# Autodesk Inventor assembly: Ensamblaje_Final
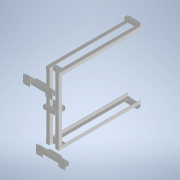
[picture p0: Inventor's stored thumbnail of the model, 180x180]
Saved by Autodesk Inventor 2020 (Build 240168000, 168)
## iProperties
Created: 2022-03-28
Part Number: Ensamblaje_Final
Document SubType Name: Assembly
Designer: aarco
Author: aarco
## Documents named in this file (8)
- C:\Users\aarco\Desktop\IDOM\REV_3\Ensamblaje_Final.iam
- C:\Users\aarco\Desktop\IDOM\REV_3\C_358_40_2.ipt
- C:\Users\aarco\Desktop\IDOM\REV_3\C_150_40_2.ipt
- C:\Users\aarco\Desktop\IDOM\REV_3\C_805_40_2.ipt
- C:\Users\aarco\Desktop\IDOM\REV_3\C_154_40_2.ipt
- C:\Users\aarco\Desktop\IDOM\REV_3\Placa_Rueda_105x85_80x60_3.ipt
- C:\Users\aarco\Desktop\IDOM\REV_3\A_992_40_4.ipt
- C:\Users\aarco\Desktop\IDOM\REV_3\C_150_40_20_2.ipt
## Components (20 placed, 7 different names)
1. C_358_40_2:1 — Rígido:16, Rígido:19, Rígido:27
2. C_358_40_2:2 — Rígido:17, Rígido:18, Rígido:26
3. C_150_40_2:1 — Rígido:1, Rígido:2
4. C_150_40_2:4 — Rígido:5
5. C_150_40_2:5 — Rígido:6
6. C_150_40_2:6 — Rígido:7
7. C_805_40_2:1 — Rígido:2, Rígido:6, Rígido:7, Rígido:22, Rígido:23
8. C_805_40_2:2 — Rígido:1, Rígido:5, Rígido:20, Rígido:21
9. C_154_40_2:1 — Rígido:24
10. C_154_40_2:2 — Rígido:25
11. Placa_Rueda_105x85_80x60_3:1 — Rígido:16
12. Placa_Rueda_105x85_80x60_3:2 — Rígido:17
13. Placa_Rueda_105x85_80x60_3:3 — Rígido:18
14. Placa_Rueda_105x85_80x60_3:4 — Rígido:19
15. A_992_40_4:1 — Rígido:20
16. A_992_40_4:2 — Rígido:22, Rígido:24
17. A_992_40_4:3 — Rígido:23, Rígido:25
18. A_992_40_4:4 — Rígido:21
19. C_150_40_20_2:1 — Rígido:26
20. C_150_40_20_2:2 — Rígido:27
## Relationships (17: WeldJoint 17)
- Rígido:1 [WeldJoint]: C_150_40_2:1 ↔ C_805_40_2:2
- Rígido:2 [WeldJoint]: C_150_40_2:1 ↔ C_805_40_2:1
- Rígido:5 [WeldJoint]: C_150_40_2:4 ↔ C_805_40_2:2
- Rígido:6 [WeldJoint]: C_150_40_2:5 ↔ C_805_40_2:1
- Rígido:7 [WeldJoint]: C_150_40_2:6 ↔ C_805_40_2:1
- Rígido:16 [WeldJoint]: C_358_40_2:1 ↔ Placa_Rueda_105x85_80x60_3:1
- Rígido:17 [WeldJoint]: C_358_40_2:2 ↔ Placa_Rueda_105x85_80x60_3:2
- Rígido:18 [WeldJoint]: C_358_40_2:2 ↔ Placa_Rueda_105x85_80x60_3:3
- Rígido:19 [WeldJoint]: C_358_40_2:1 ↔ Placa_Rueda_105x85_80x60_3:4
- Rígido:20 [WeldJoint]: C_805_40_2:2 ↔ A_992_40_4:1
- Rígido:21 [WeldJoint]: C_805_40_2:2 ↔ A_992_40_4:4
- Rígido:22 [WeldJoint]: C_805_40_2:1 ↔ A_992_40_4:2
- Rígido:23 [WeldJoint]: C_805_40_2:1 ↔ A_992_40_4:3
- Rígido:24 [WeldJoint]: C_154_40_2:1 ↔ A_992_40_4:2
- Rígido:25 [WeldJoint]: C_154_40_2:2 ↔ A_992_40_4:3
- Rígido:26 [WeldJoint]: C_358_40_2:2 ↔ C_150_40_20_2:1
- Rígido:27 [WeldJoint]: C_358_40_2:1 ↔ C_150_40_20_2:2
